# Autodesk Inventor assembly: Empaquetadora
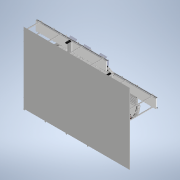
[picture p0: Inventor's stored thumbnail of the model, 180x180]
Saved by Autodesk Inventor 2022 (Build 260153000, 153)
## iProperties
Created: 2023-04-08
Part Number: Empaquetadora
Document SubType Name: Assembly
Designer: USUARIO
Author: USUARIO
## Documents named in this file (12)
- C:\Users\USUARIO\Documents\Academico\2023-I\APM\Proyecto\Gemelo Digital\Empaquetado\Empaquetadora.iam
- C:\Users\USUARIO\Documents\Academico\2023-I\APM\Proyecto\Gemelo Digital\Empaquetado\Suelo.ipt
- C:\Users\USUARIO\Documents\Academico\2023-I\APM\Proyecto\Gemelo Digital\Empaquetado\Banda I 5m\Banda_5m.iam
- C:\Users\USUARIO\Documents\Academico\2023-I\APM\Proyecto\Gemelo Digital\Empaquetado\Banda U\Banda_U.iam
- C:\Users\USUARIO\Documents\Academico\2023-I\APM\Proyecto\Gemelo Digital\Empaquetado\Banda I 3m\Banda_3m.iam
- C:\Users\USUARIO\Documents\Academico\2023-I\APM\Proyecto\Gemelo Digital\Empaquetado\Banda L\Banda_curva.iam
- C:\Users\USUARIO\Documents\Academico\2023-I\APM\Proyecto\Gemelo Digital\Empaquetado\Banda_out\Banda_Out_Cajas.iam
- C:\Users\USUARIO\Documents\Academico\2023-I\APM\Proyecto\Gemelo Digital\Empaquetado\Bandas_empaques\Bandas_separadoras.iam
- C:\Users\USUARIO\Documents\Academico\2023-I\APM\Proyecto\Gemelo Digital\Empaquetado\Caja\Caja.ipt
- C:\Users\USUARIO\Documents\Academico\2023-I\APM\Proyecto\Gemelo Digital\Empaquetado\Banda_union\Banda_union.iam
- C:\Users\USUARIO\Documents\Academico\2023-I\APM\Proyecto\Gemelo Digital\Empaquetado\Actuador\cylinder_aq232x500.iam
- C:\Users\USUARIO\Documents\Academico\2023-I\APM\Proyecto\Gemelo Digital\Empaquetado\Sensor\Sensor.iam
## Components (27 placed, 11 different names)
1. Suelo:1 — Coincidencia:1, Coincidencia:2, Nivelación:1, Coincidencia:3, Coincidencia:4, Coincidencia:5, Coincidencia:6, Coincidencia:7, Coincidencia:8, Coincidencia:9, Nivelación:2, Coincidencia:11, Coincidencia:12, Coincidencia:14, Nivelación:3
2. Banda_5m:1 [sub-assembly] — Coincidencia:1, Tangente:1, Tangente:5, Tangente:8, Tangente:9, Tangente:10, Coincidencia:24, Coincidencia:25, Coincidencia:26, Coincidencia:27, Coincidencia:28, Coincidencia:29, Tangente:15, Nivelación:4
3. Banda_U:1 [sub-assembly] — Coincidencia:2, Tangente:1, Nivelación:1, Tangente:3, Tangente:4, Tangente:5
4. Banda_3m:1 [sub-assembly] — Coincidencia:3, Tangente:3, Tangente:4, Tangente:6, Tangente:7, Tangente:11, Tangente:12, Tangente:13, Coincidencia:30, Coincidencia:31, Coincidencia:32, Coincidencia:33, Coincidencia:34, Coincidencia:35
5. Banda_curva:1 [sub-assembly] — Tangente:6, Coincidencia:4, Tangente:7, Coincidencia:23, Tangente:14
6. Banda_Out_Cajas:1 [sub-assembly] — Coincidencia:6, Nivelación:2, Coincidencia:10, Coincidencia:20, Coincidencia:21, Coincidencia:22
7. Banda_Out_Cajas:2 [sub-assembly] — Coincidencia:5, Coincidencia:16, Nivelación:3, Coincidencia:17, Coincidencia:18, Coincidencia:19
8. Bandas_separadoras:1 [sub-assembly] — Coincidencia:7, Tangente:8
9. Bandas_separadoras:2 [sub-assembly] — Coincidencia:8, Tangente:9
10. Bandas_separadoras:3 [sub-assembly] — Coincidencia:9, Tangente:10, Coincidencia:10
11. Bandas_separadoras:4 [sub-assembly] — Coincidencia:11, Tangente:11
12. Bandas_separadoras:5 [sub-assembly] — Coincidencia:12, Tangente:12
13. Bandas_separadoras:6 [sub-assembly] — Coincidencia:14, Coincidencia:16, Tangente:13
14. Caja:1 — Coincidencia:20
15. Caja:2 — Coincidencia:21
16. Caja:3 — Coincidencia:22
17. Caja:4 — Coincidencia:17
18. Caja:5 — Coincidencia:18
19. Caja:6 — Coincidencia:19
20. Banda_union:1 [sub-assembly] — Coincidencia:23, Tangente:14
21. cylinder_aq232x500:1 [sub-assembly] — Coincidencia:24, Coincidencia:27
22. cylinder_aq232x500:2 [sub-assembly] — Coincidencia:25, Coincidencia:28
23. cylinder_aq232x500:3 [sub-assembly] — Coincidencia:26, Coincidencia:29
24. cylinder_aq232x500:4 [sub-assembly] — Coincidencia:30, Coincidencia:31
25. cylinder_aq232x500:5 [sub-assembly] — Coincidencia:32, Coincidencia:33
26. cylinder_aq232x500:6 [sub-assembly] — Coincidencia:34, Coincidencia:35
27. Sensor:2 [sub-assembly] — Tangente:15, Nivelación:4
## Relationships (51: Mate 33, Tangent 14, Flush 4)
- Coincidencia:1 [Mate]: Suelo:1 ↔ Banda_5m:1
- Coincidencia:2 [Mate]: Suelo:1 ↔ Banda_U:1
- Tangente:1 (20 mm): Banda_5m:1 ↔ Banda_U:1
- Nivelación:1 [Flush]: Suelo:1 ↔ Banda_U:1
- Coincidencia:3 [Mate]: Suelo:1 ↔ Banda_3m:1
- Tangente:3 (20 mm): Banda_U:1 ↔ Banda_3m:1
- Tangente:4: Banda_U:1 ↔ Banda_3m:1
- Tangente:5: Banda_5m:1 ↔ Banda_U:1
- Tangente:6 (20 mm): Banda_3m:1 ↔ Banda_curva:1
- Coincidencia:4 [Mate]: Suelo:1 ↔ Banda_curva:1
- Tangente:7: Banda_3m:1 ↔ Banda_curva:1
- Coincidencia:5 [Mate]: Suelo:1 ↔ Banda_Out_Cajas:2
- Coincidencia:6 [Mate]: Suelo:1 ↔ Banda_Out_Cajas:1
- Coincidencia:7 [Mate]: Suelo:1 ↔ Bandas_separadoras:1
- Tangente:8: Banda_5m:1 ↔ Bandas_separadoras:1
- Coincidencia:8 [Mate]: Suelo:1 ↔ Bandas_separadoras:2
- Tangente:9: Banda_5m:1 ↔ Bandas_separadoras:2
- Coincidencia:9 [Mate]: Suelo:1 ↔ Bandas_separadoras:3
- Tangente:10: Banda_5m:1 ↔ Bandas_separadoras:3
- Nivelación:2 [Flush]: Suelo:1 ↔ Banda_Out_Cajas:1
- Coincidencia:10 [Mate] (50 mm): Banda_Out_Cajas:1 ↔ Bandas_separadoras:3
- Coincidencia:11 [Mate]: Suelo:1 ↔ Bandas_separadoras:4
- Tangente:11: Banda_3m:1 ↔ Bandas_separadoras:4
- Coincidencia:12 [Mate]: Suelo:1 ↔ Bandas_separadoras:5
- Coincidencia:14 [Mate]: Suelo:1 ↔ Bandas_separadoras:6
- Coincidencia:16 [Mate] (50 mm): Banda_Out_Cajas:2 ↔ Bandas_separadoras:6
- Nivelación:3 [Flush]: Suelo:1 ↔ Banda_Out_Cajas:2
- Tangente:12: Banda_3m:1 ↔ Bandas_separadoras:5
- Tangente:13: Banda_3m:1 ↔ Bandas_separadoras:6
- Coincidencia:17 [Mate]: Banda_Out_Cajas:2 ↔ Caja:4
- Coincidencia:18 [Mate]: Banda_Out_Cajas:2 ↔ Caja:5
- Coincidencia:19 [Mate]: Banda_Out_Cajas:2 ↔ Caja:6
- Coincidencia:20 [Mate]: Banda_Out_Cajas:1 ↔ Caja:1
- Coincidencia:21 [Mate]: Banda_Out_Cajas:1 ↔ Caja:2
- Coincidencia:22 [Mate]: Banda_Out_Cajas:1 ↔ Caja:3
- Coincidencia:23 [Mate]: Banda_curva:1 ↔ Banda_union:1
- Tangente:14: Banda_curva:1 ↔ Banda_union:1
- Coincidencia:24 [Mate]: Banda_5m:1 ↔ cylinder_aq232x500:1
- Coincidencia:25 [Mate]: Banda_5m:1 ↔ cylinder_aq232x500:2
- Coincidencia:26 [Mate]: Banda_5m:1 ↔ cylinder_aq232x500:3
- Coincidencia:27 [Mate]: Banda_5m:1 ↔ cylinder_aq232x500:1
- Coincidencia:28 [Mate]: Banda_5m:1 ↔ cylinder_aq232x500:2
- Coincidencia:29 [Mate]: Banda_5m:1 ↔ cylinder_aq232x500:3
- Coincidencia:30 [Mate]: Banda_3m:1 ↔ cylinder_aq232x500:4
- Coincidencia:31 [Mate]: Banda_3m:1 ↔ cylinder_aq232x500:4
- Coincidencia:32 [Mate]: Banda_3m:1 ↔ cylinder_aq232x500:5
- Coincidencia:33 [Mate]: Banda_3m:1 ↔ cylinder_aq232x500:5
- Coincidencia:34 [Mate]: Banda_3m:1 ↔ cylinder_aq232x500:6
- Coincidencia:35 [Mate]: Banda_3m:1 ↔ cylinder_aq232x500:6
- Tangente:15: Banda_5m:1 ↔ Sensor:2
- Nivelación:4 [Flush]: Banda_5m:1 ↔ Sensor:2
